# Autodesk Inventor assembly: Sub-Assembly 01
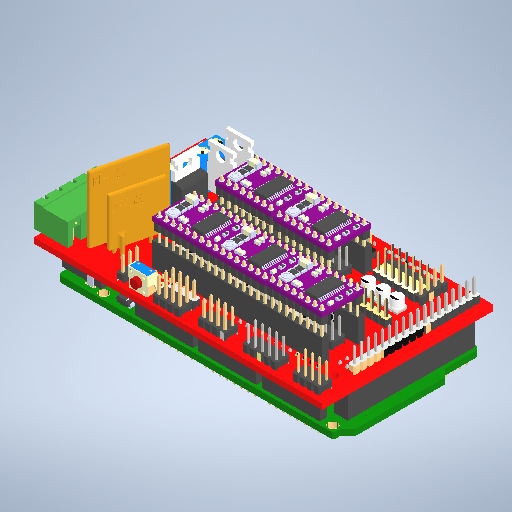
[picture p0: Inventor's stored thumbnail of the model, 512x512]
Saved by Autodesk Inventor 2025 (Build 290162000, 162)
## iProperties
Created: 2024-08-08
Part Number: Sub-Assembly 01
Document SubType Name: Assembly
Designer: PC
Author: PC
## Documents named in this file (4)
- D:\Github\CYAN\3D Model\Electronics\Sub-Assembly 01.iam
- D:\Github\CYAN\3D Model\Electronics\Shield Ramps 1.4\Shield Ramps 1.4.ipt
- D:\Github\CYAN\3D Model\Electronics\Arduino MEGA 2560\Arduino MEGA 2560.ipt
- D:\Github\CYAN\3D Model\Electronics\DRV8825\DRV8825.ipt
## Components (7 placed, 3 different names)
1. Arduino MEGA 2560:1 — Coincidencia:1
2. Shield Ramps 1.4:1 — Coincidencia:1, Coincidencia:2, Coincidencia:3, Coincidencia:4, Coincidencia:5, Coincidencia:6
3. DRV8825:3 — Coincidencia:4
4. DRV8825:4 — Coincidencia:2
5. DRV8825:5 — Coincidencia:5
6. DRV8825:6 — Coincidencia:3
7. DRV8825:8 — Coincidencia:6
## Relationships (6: Mate 6)
- Coincidencia:1 [Mate]: Arduino MEGA 2560:1 ↔ Shield Ramps 1.4:1
- Coincidencia:2 [Mate]: Shield Ramps 1.4:1 ↔ DRV8825:4
- Coincidencia:3 [Mate]: Shield Ramps 1.4:1 ↔ DRV8825:6
- Coincidencia:4 [Mate]: Shield Ramps 1.4:1 ↔ DRV8825:3
- Coincidencia:5 [Mate]: Shield Ramps 1.4:1 ↔ DRV8825:5
- Coincidencia:6 [Mate]: Shield Ramps 1.4:1 ↔ DRV8825:8
